# Autodesk Inventor assembly: topassy
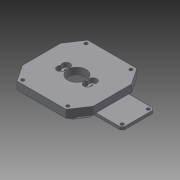
[picture p0: Inventor's stored thumbnail of the model, 180x180]
Saved by Autodesk Inventor 2018 (Build 220112000, 112)
## iProperties
Created: 2019-02-22
Part Number: topassy
Material: 一般
Document SubType Name: Assembly
Designer: ku_sk
Author: ku_sk
## Documents named in this file (3)
- E:\windows\Documents\Inventor\Content Center Files\bay shooter\parts\topassy.iam
- E:\windows\Documents\Inventor\Content Center Files\bay shooter\parts\topcover.ipt
- E:\windows\Documents\Inventor\Content Center Files\bay shooter\parts\skyrimlogo2_1_9.ipt
## Components (2 placed, 2 different names)
1. topcover:1 — メイト:1, メイト:2, メイト:3, フラッシュ:1, 角度:1
2. skyrimlogo2_1_9:1 — フラッシュ:1, 角度:1, メイト:4
## Relationships (6: Mate 4, Flush 1, Angle 1)
- メイト:1 [Mate]: topcover:1
- メイト:2 [Mate]: topcover:1
- メイト:3 [Mate]: topcover:1
- フラッシュ:1 [Flush] (1 mm): topcover:1 ↔ skyrimlogo2_1_9:1
- 角度:1 [Angle] (26.37 deg): topcover:1 ↔ skyrimlogo2_1_9:1
- メイト:4 [Mate]: skyrimlogo2_1_9:1
